# Autodesk Inventor assembly: WheelAndPocket
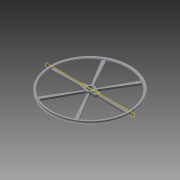
[picture p0: Inventor's stored thumbnail of the model, 180x180]
Saved by Autodesk Inventor 2014 SP1 (Build 180222100, 222)
## iProperties
Created: 2017-01-17
Part Number: WheelAndPocket
Document SubType Name: Assembly
Designer: danielsikar
Author: danielsikar
## Documents named in this file (3)
- C:\Users\danielsikar\Documents\Inventor\IoT-Trike\Assemblies\WheelAndPocket.iam
- C:\Users\danielsikar\Documents\Inventor\IoT-Trike\Parts\WheelDia190.ipt
- C:\Users\danielsikar\Documents\Inventor\IoT-Trike\Parts\ServoHornPocket.ipt
## Components (2 placed, 2 different names)
1. WheelDia190:1 — Mate:1, Mate:2, Mate:3, Mate:5
2. ServoHornPocket:1 — Mate:4, Mate:5, Mate:6
## Relationships (6: Mate 6)
- Mate:1: WheelDia190:1
- Mate:2: WheelDia190:1
- Mate:3: WheelDia190:1
- Mate:4: ServoHornPocket:1
- Mate:5: WheelDia190:1 ↔ ServoHornPocket:1
- Mate:6: ServoHornPocket:1
